# Autodesk Inventor assembly: coupler extention arm collector middle + pulleys
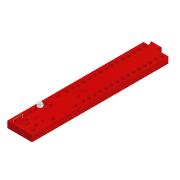
[picture p0: Inventor's stored thumbnail of the model, 180x180]
Saved by Autodesk Inventor 2020 (Build 240168000, 168)
## iProperties
Created: 2020-01-01
Part Number: coupler extention arm collector middle + pulleys
Document SubType Name: Assembly
Designer: ball
Author: ball
## Documents named in this file (5)
- C:\FTC\FTC8863CAD\2019 Robot\Delivery\extension arm\coupler extention arm collector bottom + pulleys.iam
- C:\FTC\FTC8863CAD\2019 Robot\Delivery\extension arm\Coupler extension arm short.ipt
- C:\FTC\FTC8863CAD\2019 Robot\Delivery\plastic pulley deep u.ipt
- C:\FTC\FTC8863CAD\StepLibraries\Washers\M3 FLAT WASHER.ipt
- C:\FTC\FTC8863CAD\StepLibraries\Screws\M3 x 8 SOCKET HEAD CAP SCREW.ipt
## Components (5 placed, 4 different names)
1. Coupler extension arm short:1 — Mate:6, Mate:7, Mate:8, Mate:9
2. plastic pulley deep u:1 — Mate:6, Mate:7
3. M3 FLAT WASHER:1 — Mate:8, Mate:9, Mate:10, Mate:11
4. M3 FLAT WASHER:2 — Mate:10, Mate:11, Mate:12, Mate:13
5. M3 x 8 SOCKET HEAD CAP SCREW:1 — Mate:12, Mate:13
## Relationships (8: Mate 8)
- Mate:6: Coupler extension arm short:1 ↔ plastic pulley deep u:1
- Mate:7: Coupler extension arm short:1 ↔ plastic pulley deep u:1
- Mate:8: Coupler extension arm short:1 ↔ M3 FLAT WASHER:1
- Mate:9: Coupler extension arm short:1 ↔ M3 FLAT WASHER:1
- Mate:10 (1 mm): M3 FLAT WASHER:1 ↔ M3 FLAT WASHER:2
- Mate:11: M3 FLAT WASHER:1 ↔ M3 FLAT WASHER:2
- Mate:12: M3 FLAT WASHER:2 ↔ M3 x 8 SOCKET HEAD CAP SCREW:1
- Mate:13: M3 FLAT WASHER:2 ↔ M3 x 8 SOCKET HEAD CAP SCREW:1
